# Autodesk Inventor assembly: chess board assembly 2
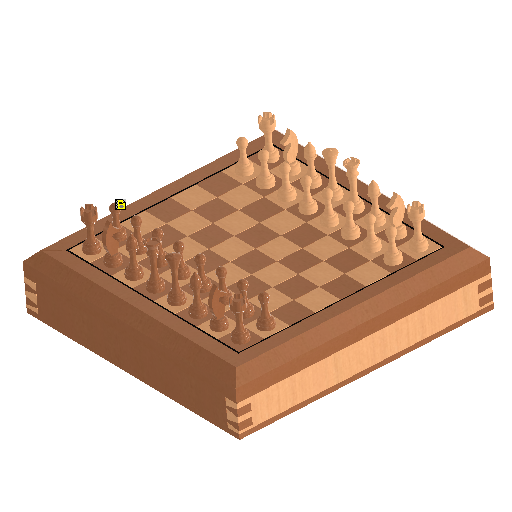
[picture p0: Inventor's stored thumbnail of the model, 512x512]
Saved by Autodesk Inventor 2025 (Build 290162000, 162)
## iProperties
Created: 2024-09-29
Part Number: chess board assembly 2
Document SubType Name: Assembly
Designer: teiko
Author: teiko
## Documents named in this file (15)
- C:\Users\teiko\OneDrive\Documents\Inventor\chess board\assembly\chess board assembly 2.iam
- C:\Users\teiko\OneDrive\Documents\Inventor\chess board\parts\box\box assembly.iam
- C:\Users\teiko\OneDrive\Documents\Inventor\chess board\parts\top\top assembly.iam
- C:\Users\teiko\OneDrive\Documents\Inventor\chess board\parts\chess pieces\pawn.ipt
- C:\Users\teiko\OneDrive\Documents\Inventor\chess board\parts\chess pieces\pawn cherry.ipt
- C:\Users\teiko\OneDrive\Documents\Inventor\chess board\parts\chess pieces\rock.ipt
- C:\Users\teiko\OneDrive\Documents\Inventor\chess board\parts\chess pieces\rock cherry.ipt
- C:\Users\teiko\OneDrive\Documents\Inventor\chess board\parts\chess pieces\knight cherry.ipt
- C:\Users\teiko\OneDrive\Documents\Inventor\chess board\parts\chess pieces\knight.ipt
- C:\Users\teiko\OneDrive\Documents\Inventor\chess board\parts\chess pieces\bishop.ipt
- C:\Users\teiko\OneDrive\Documents\Inventor\chess board\parts\chess pieces\bishop cherry.ipt
- C:\Users\teiko\OneDrive\Documents\Inventor\chess board\parts\chess pieces\king walnut.ipt
- C:\Users\teiko\OneDrive\Documents\Inventor\chess board\parts\chess pieces\king cherry 2.ipt
- C:\Users\teiko\OneDrive\Documents\Inventor\chess board\parts\chess pieces\queen.ipt
- C:\Users\teiko\OneDrive\Documents\Inventor\chess board\parts\chess pieces\queen cherry.ipt
## Components (35 placed, 14 different names)
1. box assembly:1 [sub-assembly] — Mate:1, Flush:1, Mate:2, Mate:3, Mate:4, Mate:5
2. top assembly:1 [sub-assembly] — Mate:1, Flush:1, Mate:5, Mate:6, Mate:10, Mate:11, Flush:4, Mate:14, Flush:5, Mate:15, Flush:6, Mate:16, Mate:17, Flush:7, Mate:27, Mate:28, Mate:29, Mate:32, Flush:8, Flush:9, Flush:10, Mate:36, Mate:37, Mate:40, Mate:41, Mate:42, Flush:12, Mate:46, Mate:47, Flush:14, Mate:50, Flush:15, Flush:16, Mate:54, Flush:18, Mate:56, Mate:60, Mate:61, Flush:20
3. top assembly:2 [sub-assembly] — Mate:2, Mate:3, Mate:4, Mate:9, Mate:12, Mate:13, Mate:18, Mate:19, Mate:20, Mate:21, Mate:22, Mate:23, Mate:24, Mate:25, Mate:26, Mate:30, Mate:31, Flush:11, Mate:33, Mate:34, Mate:35, Mate:38, Mate:39, Mate:43, Flush:13, Mate:44, Mate:45, Mate:48, Mate:49, Mate:51, Flush:17, Mate:52, Mate:53, Mate:57, Flush:19, Mate:58, Mate:59, Mate:62, Mate:63
4. pawn:1 — Mate:6, Flush:4, Mate:27
5. pawn cherry:1 — Mate:9, Mate:18, Mate:19
6. pawn:2 — Mate:10, Mate:14, Flush:5
7. pawn:3 — Mate:11, Mate:15, Flush:6
8. pawn cherry:2 — Mate:13, Mate:22, Mate:23
9. pawn cherry:3 — Mate:12, Mate:20, Mate:21
10. rock:1 — Mate:28, Mate:32, Flush:8
11. rock:2 — Mate:29, Flush:9, Flush:10
12. rock cherry:1 — Mate:31, Mate:34, Mate:35
13. rock cherry:2 — Mate:30, Flush:11, Mate:33
14. knight cherry:1 — Mate:38, Mate:43, Flush:13
15. knight cherry:2 — Mate:39, Mate:44, Mate:45
16. knight:1 — Mate:36, Mate:40, Mate:41
17. knight:2 — Mate:37, Mate:42, Flush:12
18. bishop:1 — Mate:47, Flush:15, Flush:16
19. bishop:2 — Mate:46, Flush:14, Mate:50
20. bishop cherry:1 — Mate:49, Mate:52, Mate:53
21. bishop cherry:2 — Mate:48, Mate:51, Flush:17
22. king walnut:1 — Mate:54, Flush:18, Mate:56
23. king cherry 2:1 — Mate:57, Flush:19, Mate:58
24. queen:1 — Mate:60, Mate:61, Flush:20
25. queen cherry:1 — Mate:59, Mate:62, Mate:63
26. pawn cherry:4 — Mate:24, Mate:25, Mate:26
27. pawn:4 — Mate:16, Mate:17, Flush:7
28. pawn cherry:5
29. pawn:5
30. pawn cherry:6
31. pawn:6
32. pawn cherry:7
33. pawn:7
34. pawn cherry:8
35. pawn:8
## Component patterns: (5 elements, first: pawn cherry:4 + pawn:4)
## Relationships (78: Mate 60, Flush 18)
- Mate:1: box assembly:1 ↔ top assembly:1
- Flush:1: box assembly:1 ↔ top assembly:1
- Mate:2: box assembly:1 ↔ top assembly:2
- Mate:3: box assembly:1 ↔ top assembly:2
- Mate:4: box assembly:1 ↔ top assembly:2
- Mate:5: box assembly:1 ↔ top assembly:1
- Mate:6: top assembly:1 ↔ pawn:1
- Mate:9: top assembly:2 ↔ pawn cherry:1
- Mate:10: top assembly:1 ↔ pawn:2
- Mate:11: top assembly:1 ↔ pawn:3
- Mate:12: top assembly:2 ↔ pawn cherry:3
- Mate:13: top assembly:2 ↔ pawn cherry:2
- Flush:4 (125 mm): top assembly:1 ↔ pawn:1
- Mate:14 (-125 mm): top assembly:1 ↔ pawn:2
- Flush:5 (125 mm): top assembly:1 ↔ pawn:2
- Mate:15 (-175 mm): top assembly:1 ↔ pawn:3
- Flush:6 (125 mm): top assembly:1 ↔ pawn:3
- Mate:16: top assembly:1 ↔ pawn:4
- Mate:17 (-125 mm): top assembly:1 ↔ pawn:4
- Flush:7 (225 mm): top assembly:1 ↔ pawn:4
- Mate:18 (-125 mm): top assembly:2 ↔ pawn cherry:1
- Mate:19 (-75 mm): top assembly:2 ↔ pawn cherry:1
- Mate:20 (-125 mm): top assembly:2 ↔ pawn cherry:3
- Mate:21 (-125 mm): top assembly:2 ↔ pawn cherry:3
- Mate:22 (-125 mm): top assembly:2 ↔ pawn cherry:2
- Mate:23 (-175 mm): top assembly:2 ↔ pawn cherry:2
- Mate:24: top assembly:2 ↔ pawn cherry:4
- Mate:25 (-125 mm): top assembly:2 ↔ pawn cherry:4
- Mate:26 (-225 mm): top assembly:2 ↔ pawn cherry:4
- Mate:27 (-75 mm): top assembly:1 ↔ pawn:1
- Mate:28: top assembly:1 ↔ rock:1
- Mate:29: top assembly:1 ↔ rock:2
- Mate:30: top assembly:2 ↔ rock cherry:2
- Mate:31: top assembly:2 ↔ rock cherry:1
- Mate:32 (-75 mm): top assembly:1 ↔ rock:1
- Flush:8 (75 mm): top assembly:1 ↔ rock:1
- Flush:9 (75 mm): top assembly:1 ↔ rock:2
- Flush:10 (75 mm): top assembly:1 ↔ rock:2
- Flush:11 (75 mm): top assembly:2 ↔ rock cherry:2
- Mate:33 (-75 mm): top assembly:2 ↔ rock cherry:2
- Mate:34 (-75 mm): top assembly:2 ↔ rock cherry:1
- Mate:35 (-75 mm): top assembly:2 ↔ rock cherry:1
- Mate:36: top assembly:1 ↔ knight:1
- Mate:37: top assembly:1 ↔ knight:2
- Mate:38: top assembly:2 ↔ knight cherry:1
- Mate:39: top assembly:2 ↔ knight cherry:2
- Mate:40 (-75 mm): top assembly:1 ↔ knight:1
- Mate:41 (-125 mm): top assembly:1 ↔ knight:1
- Mate:42 (-75 mm): top assembly:1 ↔ knight:2
- Flush:12 (125 mm): top assembly:1 ↔ knight:2
- Mate:43 (-75 mm): top assembly:2 ↔ knight cherry:1
- Flush:13 (125 mm): top assembly:2 ↔ knight cherry:1
- Mate:44 (-75 mm): top assembly:2 ↔ knight cherry:2
- Mate:45 (-125 mm): top assembly:2 ↔ knight cherry:2
- Mate:46: top assembly:1 ↔ bishop:2
- Mate:47: top assembly:1 ↔ bishop:1
- Mate:48: top assembly:2 ↔ bishop cherry:2
- Mate:49: top assembly:2 ↔ bishop cherry:1
- Flush:14 (75 mm): top assembly:1 ↔ bishop:2
- Mate:50 (-175 mm): top assembly:1 ↔ bishop:2
- Flush:15 (175 mm): top assembly:1 ↔ bishop:1
- Flush:16 (75 mm): top assembly:1 ↔ bishop:1
- Mate:51 (-75 mm): top assembly:2 ↔ bishop cherry:2
- Flush:17 (175 mm): top assembly:2 ↔ bishop cherry:2
- Mate:52 (-175 mm): top assembly:2 ↔ bishop cherry:1
- Mate:53 (-75 mm): top assembly:2 ↔ bishop cherry:1
- Mate:54: top assembly:1 ↔ king walnut:1
- Flush:18 (75 mm): top assembly:1 ↔ king walnut:1
- Mate:56 (-225 mm): top assembly:1 ↔ king walnut:1
- Mate:57: top assembly:2 ↔ king cherry 2:1
- Flush:19 (225 mm): top assembly:2 ↔ king cherry 2:1
- Mate:58 (-75 mm): top assembly:2 ↔ king cherry 2:1
- Mate:59: top assembly:2 ↔ queen cherry:1
- Mate:60: top assembly:1 ↔ queen:1
- Mate:61 (-75 mm): top assembly:1 ↔ queen:1
- Flush:20 (225 mm): top assembly:1 ↔ queen:1
- Mate:62 (-75 mm): top assembly:2 ↔ queen cherry:1
- Mate:63 (-225 mm): top assembly:2 ↔ queen cherry:1
